# Autodesk Inventor assembly: Finalassembly
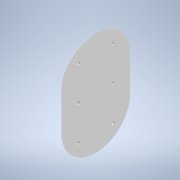
[picture p0: Inventor's stored thumbnail of the model, 180x180]
Saved by Autodesk Inventor 2022 (Build 260153000, 153)
## iProperties
Created: 2022-04-25
Part Number: Finalassembly
Document SubType Name: Assembly
Designer: Bruger
Author: Bruger
## Documents named in this file (4)
- C:\Users\Bruger\Desktop\SDU\Civilingeniør\2. Semester\Project in Advanced Robotics\Git\Finalassembly.iam
- C:\Users\Bruger\Desktop\SDU\Civilingeniør\2. Semester\Project in Advanced Robotics\Git\3DPrintShapeStraightEdge1.ipt
- C:\Users\Bruger\Desktop\SDU\Civilingeniør\2. Semester\Project in Advanced Robotics\Git\3DPrintShapeStraightEdge2.ipt
- C:\Users\Bruger\Desktop\SDU\Civilingeniør\2. Semester\Project in Advanced Robotics\Git\3DPrintShapeCorner.ipt
## Components (6 placed, 3 different names)
1. 3DPrintShapeCorner:1 — Rigid:2, Rigid:3
2. 3DPrintShapeCorner:2 — Rigid:3
3. 3DPrintShapeCorner:3 — Rigid:5
4. 3DPrintShapeCorner:4 — Rigid:4
5. 3DPrintShapeStraightEdge1:1 — Rigid:1, Rigid:2, Rigid:4
6. 3DPrintShapeStraightEdge2:1 — Rigid:1, Rigid:5
## Relationships (5: WeldJoint 5)
- Rigid:1 [WeldJoint]: 3DPrintShapeStraightEdge1:1 ↔ 3DPrintShapeStraightEdge2:1
- Rigid:2 [WeldJoint]: 3DPrintShapeCorner:1 ↔ 3DPrintShapeStraightEdge1:1
- Rigid:3 [WeldJoint]: 3DPrintShapeCorner:1 ↔ 3DPrintShapeCorner:2
- Rigid:4 [WeldJoint]: 3DPrintShapeCorner:4 ↔ 3DPrintShapeStraightEdge1:1
- Rigid:5 [WeldJoint]: 3DPrintShapeCorner:3 ↔ 3DPrintShapeStraightEdge2:1
